# Autodesk Inventor assembly: Foot
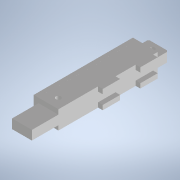
[picture p0: Inventor's stored thumbnail of the model, 180x180]
Saved by Autodesk Inventor 2020 (Build 240168000, 168)
## iProperties
Created: 2019-12-19
Part Number: Foot
Document SubType Name: Assembly
Designer: damien
Author: damien
## Documents named in this file (4)
- D:\fablab\save\Foot.iam
- D:\fablab\save\graduated_foot_03.ipt
- D:\fablab\save\rail.ipt
- D:\fablab\save\cover.ipt
## Components (5 placed, 3 different names)
1. graduated_foot_03:1 — Placage:1, Affleurement:1, Affleurement:2, Placage:2, Affleurement:8
2. graduated_foot_03:2 — Placage:1, Affleurement:1, Affleurement:2, Placage:3, Affleurement:9
3. rail:1 — Placage:3, Affleurement:3, Affleurement:4, Affleurement:7, Affleurement:9
4. rail:2 — Placage:2, Affleurement:3, Affleurement:4, Affleurement:6, Affleurement:8, Placage:4
5. cover:1 — Affleurement:6, Affleurement:7, Placage:4
## Relationships (12: Flush 8, Mate 4)
- Placage:1 [Mate]: graduated_foot_03:1 ↔ graduated_foot_03:2
- Affleurement:1 [Flush]: graduated_foot_03:1 ↔ graduated_foot_03:2
- Affleurement:2 [Flush]: graduated_foot_03:1 ↔ graduated_foot_03:2
- Placage:2 [Mate]: graduated_foot_03:1 ↔ rail:2
- Placage:3 [Mate]: graduated_foot_03:2 ↔ rail:1
- Affleurement:3 [Flush]: rail:1 ↔ rail:2
- Affleurement:4 [Flush]: rail:1 ↔ rail:2
- Affleurement:6 [Flush]: rail:2 ↔ cover:1
- Affleurement:7 [Flush]: rail:1 ↔ cover:1
- Affleurement:8 [Flush]: graduated_foot_03:1 ↔ rail:2
- Placage:4 [Mate]: rail:2 ↔ cover:1
- Affleurement:9 [Flush] (-42.9 mm): graduated_foot_03:2 ↔ rail:1
